# Autodesk Inventor assembly: Full Extension Ball bearing Slide
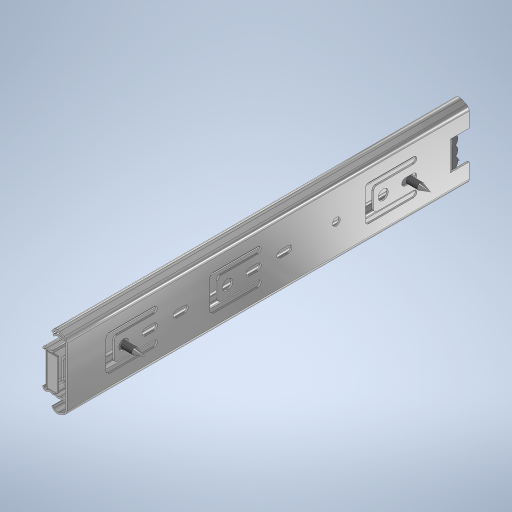
[picture p0: Inventor's stored thumbnail of the model, 512x512]
Saved by Autodesk Inventor 2024 (Build 280153000, 153)
## iProperties
Created: 2013-11-19
Part Number: Full Extension Ball bearing Slide
Document SubType Name: Assembly
Designer: SauliusD
Description: Full Extension Ball bearing Slide
Author: SauliusD
## Documents named in this file (6)
- C:\W4INV 2024 Design\iBOX LIBRARY\Drawers\Full Pull Drawer\Parts\Full Extension Ball bearing Slide.iam
- C:\W4INV 2024 Design\iBOX LIBRARY\Drawers\Full Pull Drawer\Parts\Outer Slider Guide.ipt
- C:\W4INV 2024 Design\iBOX LIBRARY\Drawers\Full Pull Drawer\Parts\Secondary Slider Guide.ipt
- C:\W4INV 2024 Design\iBOX LIBRARY\Drawers\Full Pull Drawer\Parts\Inner Slider Guide.ipt
- C:\W4INV 2024 Design\iBOX LIBRARY\Drawers\Full Pull Drawer\Parts\Bumper.ipt
- C:\W4INV 2024 Design\iBOX LIBRARY\Drawers\Full Pull Drawer\Parts\Screw 1.ipt
## Components (8 placed, 5 different names)
1. Outer Slider Guide:1 — Insert:2, Mate:1, Mate:2
2. Secondary Slider Guide:1
3. Inner Slider Guide:1 — Insert:1
4. Bumper:1
5. Screw 1:1
6. Screw 1:2 — Insert:1
7. Screw 1:3 — Insert:2
8. Screw 1:4 — Mate:1, Mate:2
## Relationships (4: Insert 2, Mate 2)
- Insert:1: Inner Slider Guide:1 ↔ Screw 1:2
- Insert:2: Outer Slider Guide:1 ↔ Screw 1:3
- Mate:1: Outer Slider Guide:1 ↔ Screw 1:4
- Mate:2: Outer Slider Guide:1 ↔ Screw 1:4
